# Autodesk Inventor assembly: assembly-pcb
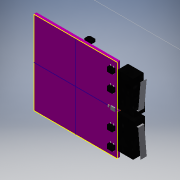
[picture p0: Inventor's stored thumbnail of the model, 180x180]
Saved by Autodesk Inventor 2016 (Build 200138000, 138)
## iProperties
Created: 2016-01-29
Part Number: assembly-pcb
Document SubType Name: Assembly
Designer: jferner
Author: jferner
## Documents named in this file (7)
- C:\dev\minirobot\mechanical\assembly-pcb.iam
- C:\dev\minirobot\mechanical\pcb.ipt
- C:\dev\minirobot\mechanical\SS-5GL-F.ipt
- C:\dev\minirobot\mechanical\QRE1113GR.ipt
- C:\dev\minirobot\mechanical\TCS3472.ipt
- C:\dev\minirobot\mechanical\LW-Q38E-Q100-3K6L-1.ipt
- C:\dev\minirobot\mechanical\QRE1113.ipt
## Components (11 placed, 6 different names)
1. pcb:1 — Mate:1, Mate:2, Mate:3, Mate:4, Flush:1, Flush:2, Mate:6, Mate:7, Mate:9, Mate:10, Flush:3, Flush:6, Flush:7, Mate:12, Mate:13, Mate:14, Mate:15, Flush:8, Flush:9, Mate:16, Mate:17, Mate:18, Mate:19, Mate:20, Mate:21, Flush:10, Flush:11, Flush:12, Flush:13
2. SS-5GL-F:1 — Mate:1, Mate:3, Flush:2
3. SS-5GL-F:2 — Mate:2, Mate:4, Flush:1
4. QRE1113GR:1 — Mate:6, Flush:3, Mate:13
5. QRE1113GR:2 — Mate:7, Flush:6, Mate:12
6. TCS3472:1 — Mate:9, Flush:7, Mate:11, Mate:18
7. LW-Q38E-Q100-3K6L-1:1 — Mate:10, Mate:11, Mate:19
8. QRE1113GR:6 — Mate:15, Flush:9, Mate:17
9. QRE1113GR:7 — Mate:14, Flush:8, Mate:16
10. QRE1113:1 — Mate:20, Flush:11, Flush:12
11. QRE1113:2 — Mate:21, Flush:10, Flush:13
## Relationships (30: Mate 19, Flush 11)
- Mate:1: pcb:1 ↔ SS-5GL-F:1
- Mate:2: pcb:1 ↔ SS-5GL-F:2
- Mate:3: pcb:1 ↔ SS-5GL-F:1
- Mate:4: pcb:1 ↔ SS-5GL-F:2
- Flush:1 (13 mm): pcb:1 ↔ SS-5GL-F:2
- Flush:2 (13 mm): pcb:1 ↔ SS-5GL-F:1
- Mate:6: pcb:1 ↔ QRE1113GR:1
- Mate:7: pcb:1 ↔ QRE1113GR:2
- Mate:9: pcb:1 ↔ TCS3472:1
- Mate:10: pcb:1 ↔ LW-Q38E-Q100-3K6L-1:1
- Flush:3 (1 mm): pcb:1 ↔ QRE1113GR:1
- Flush:6 (-1 mm): pcb:1 ↔ QRE1113GR:2
- Flush:7 (-1 mm): pcb:1 ↔ TCS3472:1
- Mate:11 (1 mm): TCS3472:1 ↔ LW-Q38E-Q100-3K6L-1:1
- Mate:12 (8.65 mm): pcb:1 ↔ QRE1113GR:2
- Mate:13 (18.65 mm): pcb:1 ↔ QRE1113GR:1
- Mate:14: pcb:1 ↔ QRE1113GR:7
- Mate:15: pcb:1 ↔ QRE1113GR:6
- Flush:8 (-1 mm): pcb:1 ↔ QRE1113GR:7
- Flush:9 (1 mm): pcb:1 ↔ QRE1113GR:6
- Mate:16 (8.65 mm): pcb:1 ↔ QRE1113GR:7
- Mate:17 (18.65 mm): pcb:1 ↔ QRE1113GR:6
- Mate:18 (-1 mm): pcb:1 ↔ TCS3472:1
- Mate:19 (-0.8 mm): pcb:1 ↔ LW-Q38E-Q100-3K6L-1:1
- Mate:20: pcb:1 ↔ QRE1113:1
- Mate:21: pcb:1 ↔ QRE1113:2
- Flush:10: pcb:1 ↔ QRE1113:2
- Flush:11: pcb:1 ↔ QRE1113:1
- Flush:12 (18.5 mm): pcb:1 ↔ QRE1113:1
- Flush:13 (18.5 mm): pcb:1 ↔ QRE1113:2
## Named parameters: QRE1113GR_x = 2.7 mm, QRE1113GR_y = 3.4 mm, TCS3472_x = 2 mm, TCS3472_y = 2.4 mm, LWQ38EQ1003K6L1_x = 0.8 mm, LWQ38EQ1003K6L1_y = 1.6 mm
